# Autodesk Inventor assembly: 3. P+K+O+PCB+Bateria
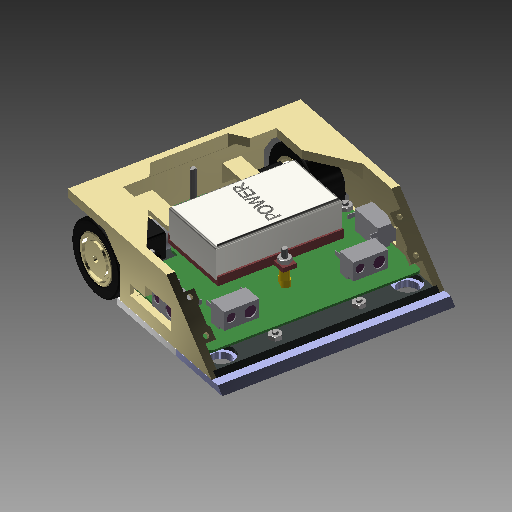
[picture p0: Inventor's stored thumbnail of the model, 512x512]
Saved by Autodesk Inventor 2017 (Build 210142000, 142)
## iProperties
Created: 2016-11-21
Part Number: 3. P+K+O+PCB+Bateria
Document SubType Name: Assembly
Designer: Shichi
Author: Shichi
## Documents named in this file (4)
- E:\h3fty\H3FTY\Model\3. P+K+O+PCB+Bateria.iam
- C:\Users\Shichi\Documents\Inventor\Content Center Files\R2017\en-US\AS 1112 (2)\AS 1112 - M2,5  Type 5.ipt
- E:\h3fty\H3FTY\Model\2. P+K+O+PCB.iam
- E:\h3fty\H3FTY\Model\Bateria\Bateria+Podkladka.iam
## Components (3 placed, 3 different names)
1. 2. P+K+O+PCB:1 [sub-assembly] — Insert:1, Insert:2
2. Bateria+Podkladka:1 [sub-assembly] — Insert:1, Insert:2, Insert:3
3. AS 1112 (2) - Metric M2,5  Type 5:1 — Insert:3
## Relationships (3: Insert 3)
- Insert:1: 2. P+K+O+PCB:1 ↔ Bateria+Podkladka:1
- Insert:2: 2. P+K+O+PCB:1 ↔ Bateria+Podkladka:1
- Insert:3: Bateria+Podkladka:1 ↔ AS 1112 (2) - Metric M2,5  Type 5:1
